# Autodesk Inventor assembly: Peli 1300
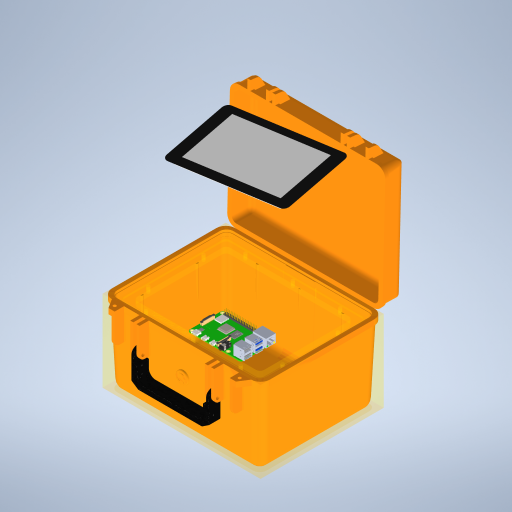
[picture p0: Inventor's stored thumbnail of the model, 512x512]
Saved by Autodesk Inventor 2023.1 (Build 271208000, 208)
## iProperties
Created: 2021-11-22
Part Number: Peli 1300
Description: STEP AP214
Document SubType Name: Assembly
Designer: Charlie Kendall
Sending System: SolidWorks 2018
Preprocessor: SwSTEP 2.0
Title: Peli 1300.STEP
Revision Number: ANY
## Documents named in this file (7)
- C:\Users\Charlie Kendall\Documents\Field Computer\Field Computer.iam
- C:\Users\Charlie Kendall\Documents\Field Computer\Case and Bezel\1300-CASE-BOT.ipt
- C:\Users\Charlie Kendall\Documents\Field Computer\Case and Bezel\1300-CASE-TOP.ipt
- C:\Users\Charlie Kendall\Documents\Field Computer\Case and Bezel\handle.ipt
- C:\Users\Charlie Kendall\Documents\Field Computer\Mainboard\Raspberry Pi 4 Model B.iam
- C:\Users\Charlie Kendall\Documents\Field Computer\Screen\Raspberry_Pi_Touch_Display.iam
- C:\Users\Charlie Kendall\Documents\Field Computer\Case and Bezel\1300-CASE-PF.ipt
## Components (6 placed, 6 different names)
1. 1300-CASE-BOT_1 — Mate:1, Flush:1, Flush:2, Flush:3, Mate:2, Mate:3, Mate:4, Flush:4, Flush:5, Flush:6, Flush:7
2. 1300-CASE-TOP_2 — Mate:4, Flush:4
3. handle_3 — Mate:2, Mate:3
4. Raspberry Pi 4 Model B:1 [sub-assembly]
5. Raspberry_Pi_Touch_Display:1 [sub-assembly]
6. 1300-CASE-PF:1 — Flush:5, Flush:6, Flush:7
## Relationships (11: Flush 7, Mate 4)
- Mate:1: 1300-CASE-BOT_1
- Flush:1: 1300-CASE-BOT_1
- Flush:2: 1300-CASE-BOT_1
- Flush:3: 1300-CASE-BOT_1
- Mate:2: 1300-CASE-BOT_1 ↔ handle_3
- Mate:3: 1300-CASE-BOT_1 ↔ handle_3
- Mate:4: 1300-CASE-BOT_1 ↔ 1300-CASE-TOP_2
- Flush:4: 1300-CASE-BOT_1 ↔ 1300-CASE-TOP_2
- Flush:5: 1300-CASE-BOT_1 ↔ 1300-CASE-PF:1
- Flush:6: 1300-CASE-BOT_1 ↔ 1300-CASE-PF:1
- Flush:7: 1300-CASE-BOT_1 ↔ 1300-CASE-PF:1
